# Autodesk Inventor assembly: Clutch Concept
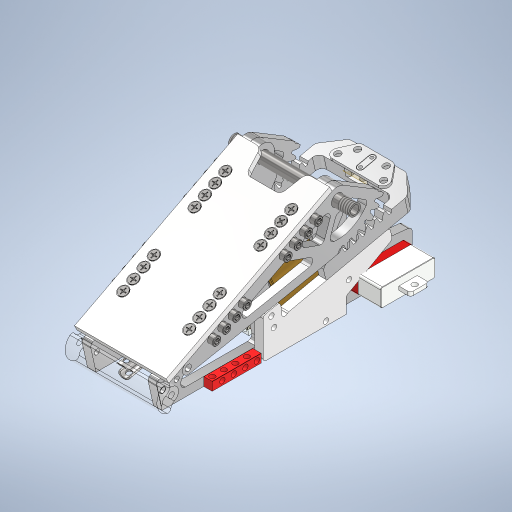
[picture p0: Inventor's stored thumbnail of the model, 512x512]
Saved by Autodesk Inventor 2023.4 (Build 274418000, 418)
## iProperties
Created: 2024-02-03
Part Number: Clutch Concept
Document SubType Name: Assembly
Designer: Nathan Cai
Mass: 1134.93 g
Surface Area: 3804.81 cm^2
Volume: 547.921 cm^3
Density: 2.07134 g/cm^3
Author: Nathan Cai
## Documents named in this file (35)
- E:\Documents\Inventor\Bleep V1.3\Clutch Concept.iam
- E:\Documents\Inventor\Bleep V1.3\Flywheel.ipt
- E:\Documents\Inventor\Bleep V1.3\Thrust Bearing.ipt
- E:\Documents\Inventor\Bleep V1.3\BB 13x19x4.ipt
- E:\Documents\Inventor\Bleep V1.3\Cup.ipt
- E:\Documents\Inventor\Bleep V1.3\1561T741_Stacked Wave Disc Spring\1561T741_Stacked Wave Disc Spring.ipt
- E:\Documents\Inventor\Bleep V1.3\AKK RS2205 2300KV\AKK RS2205 2300KV.iam
- E:\Documents\Inventor\Bleep V1.3\Nut Strip 2x1 - 4-40.ipt
- E:\Documents\Inventor\Bleep V1.3\BB 37mm x 30mm x 4mm.ipt
- E:\Documents\Inventor\Bleep V1.3\Motor Plate.ipt
- E:\Documents\Inventor\Bleep V1.3\Uprights.ipt
- E:\Documents\Inventor\Bleep V1.3\Nut Strip 4x4 - 4-40.ipt
- E:\Documents\Inventor\Bleep V1.3\5172T23_Metal Gear - 20 Degree Pressure Angle\5172T23_Metal Gear - 20 Degree Pressure Angle.ipt
- E:\Documents\Inventor\Bleep V1.3\BB .25x.5x.1875 - Flangeless.ipt
- E:\Documents\Inventor\Content Center Files\R2023\en-US\ANSI B18.3(13)\ANSI B18.3 - 4-40 UNC - 0.375(22).ipt
- E:\Documents\Inventor\Bleep V1.3\Lever.ipt
- E:\Documents\Inventor\Bleep V1.3\Part1\Part1.ipt
- E:\Documents\Inventor\Bleep V1.3\Cam - Lever.ipt
- E:\Documents\Inventor\Bleep V1.3\Cam - Shell.ipt
- E:\Documents\Inventor\Bleep V1.3\BB 3x7x3.ipt
- E:\Documents\Inventor\Bleep V1.3\Ramp.ipt
- E:\Documents\Inventor\Bleep V1.3\Lever - Copy.ipt
- E:\Documents\Inventor\Bleep V1.3\Brace.ipt
- E:\Documents\Inventor\Bleep V1.3\BB 3x7x3 - Copy.ipt
- E:\Documents\Inventor\Bleep V1.3\Shaft - Arms.ipt
- E:\Documents\Inventor\Bleep V1.3\Shaft - Flywheel C.ipt
- E:\Documents\Inventor\Bleep V1.3\Clutch C.ipt
- E:\Documents\Inventor\Bleep V1.3\Spring Mount.ipt
- E:\Documents\Inventor\Bleep V1.3\Spring Spool.ipt
- E:\Documents\Inventor\Bleep V1.3\Collar.ipt
- E:\Documents\Inventor\Content Center Files\R2023\en-US\ANSI B18.6.3(12)\ANSI B18.6.3 - 4-40 UNC - 0.375(15_).ipt
- E:\Documents\Inventor\Bleep V1.3\Front Bumper.ipt
- E:\Documents\Inventor\Bleep V1.3\Rack - Slot.ipt
- E:\Documents\Inventor\Bleep V1.3\Pin Cap - Slot.ipt
- E:\Documents\Inventor\Bleep V1.3\Export\STL\Lever Spacer.ipt
## Components (85 placed, 34 different names)
1. Front Bumper:1 — Angle:5, Mate:464, Mate:465
2. Pin Cap - Slot:1 — Mate:459, Mate:460, Mate:461
3. Lever Spacer:1 — Mate:462, Mate:463
4. Flywheel:1 — Mate:37, Flush:102, Mate:104, Mate:105, Mate:275, Mate:309
5. Shaft - Flywheel C:1 — Mate:306, Mate:307, Mate:308, Mate:310, Mate:311, Mate:312, Mate:313, Mate:314, Mate:315, Angle:4, Mate:319, Mate:321, Mate:324
6. Shaft - Arms:1 — Mate:257, Flush:118
7. Clutch C:1 — Mate:308, Angle:4
8. Rack - Slot:1 — Angle:1, Angle:3, Rotation/Translation:1, Mate:315, Mate:313, Mate:314, Mate:459, Mate:460, Mate:461
9. Cup:1 — Mate:26, Mate:27, Angle:1, Tangent:1
10. AKK RS2205 2300KV:1 [sub-assembly] — Mate:37, Flush:102, Mate:426
11. Motor Plate:1 — Mate:106, Mate:107, Mate:128, Mate:129, Mate:131, Mate:132, Mate:134, Mate:136, Flush:106, Mate:144, Mate:145, Mate:146, Mate:147, Mate:148, Mate:149, Mate:150, Mate:151, Mate:152, Mate:153, Mate:154, Mate:155, Mate:156, Mate:157, Mate:158, Mate:159, Flush:149, Mate:426
12. 1561T741_Stacked Wave Disc Spring:1 — Mate:311, Mate:312
13. Spring Mount:1 — Mate:316, Flush:149, Mate:317, Mate:320
14. Thrust Bearing:1 — Mate:319, Mate:320, Mate:322
15. Spring Spool:1 — Mate:321, Mate:322, Mate:325
16. Collar:1 — Mate:324, Mate:325
17. Uprights:1 — Mate:128, Mate:130, Flush:103, Flush:104, Mate:133, Mate:138, Mate:141, Flush:107, Mate:168, Mate:169, Mate:229, Mate:230, Flush:110, Mate:257, Mate:266, Mate:267, Mate:268, Mate:269, Flush:125, Mate:317, Mate:289, Mate:363, Angle:6, Angle:7
18. Uprights:2 — Flush:103, Mate:132, Flush:104, Mate:135, Mate:137, Mate:139, Mate:140, Mate:226, Mate:228, Flush:111, Mate:263, Mate:264, Mate:270, Mate:271, Flush:124, Mate:292, Mate:362, Angle:5, Mate:464, Mate:465, Mate:466, Mate:467, Mate:468
19. Brace:1 — Mate:226, Mate:228, Flush:111, Mate:292
20. Brace:2 — Mate:229, Mate:230, Flush:110, Mate:289
21. Nut Strip 4x4 - 4-40:1 — Mate:129, Mate:130, Mate:131, Mate:133, Mate:316
22. Nut Strip 4x4 - 4-40:2 — Mate:134, Mate:135, Mate:136, Mate:137
23. 5172T23_Metal Gear - 20 Degree Pressure Angle:1 — Mate:138, Mate:141, Flush:105, Angle:3, Mate:198, Mate:199, Mate:200, Mate:201, Mate:202, Mate:203, Mate:204, Rotation/Translation:1, Flush:118, Mate:369, Mate:427, Mate:428, Mate:429, Mate:430, Mate:431, Mate:432, Mate:433, Mate:434, Mate:435, Mate:436, Mate:437, Mate:438, Mate:439, Mate:440, Mate:441, Mate:442
24. 5172T23_Metal Gear - 20 Degree Pressure Angle:2 — Mate:139, Mate:140, Flush:105, Mate:192, Mate:193, Mate:194, Mate:195, Mate:196, Mate:197, Flush:150, Mate:443, Mate:444, Mate:445, Mate:446, Mate:447, Mate:448, Mate:449, Mate:450, Mate:451, Mate:452, Mate:453, Mate:454, Mate:455, Mate:456, Mate:457, Mate:458
25. BB .25x.5x.1875 - Flangeless:1 — Flush:106, Mate:310
26. Lever:1 — Mate:168, Mate:169, Tangent:1, Mate:181, Mate:182, Mate:190, Mate:326
27. Lever - Copy:1
28. Part1:1 — Mate:179, Mate:180, Angle:6, Angle:7, Mate:466, Mate:467, Mate:468
29. Cam - Lever:1 — Mate:177, Mate:178
30. Cam - Shell:1 — Mate:177, Mate:178, Mate:179, Mate:180
31. BB 3x7x3:1 — Mate:181, Mate:182
32. BB 3x7x3:2 — Mate:462, Mate:463
33. BB 3x7x3 - Copy:1 — Mate:190, Mate:326
34. BB 13x19x4:1 — Mate:26, Mate:27
35. BB 37mm x 30mm x 4mm:1 — Mate:104, Mate:105, Mate:106, Mate:107
36. BB .25x.5x.1875 - Flangeless:2 — Mate:275, Mate:306, Mate:307, Mate:309
37. Ramp:1 — Mate:204, Flush:150, Mate:369, Mate:370, Mate:371, Mate:372, Mate:373, Mate:374, Mate:375, Mate:376, Mate:377, Mate:378, Mate:379, Mate:380, Mate:381, Mate:382, Mate:383, Mate:384, Mate:385
38. Nut Strip 4x4 - 4-40:3 — Mate:192, Mate:193, Mate:194
39. Nut Strip 4x4 - 4-40:5 — Mate:199, Mate:200, Mate:201
40. Nut Strip 4x4 - 4-40:6 — Mate:198, Mate:202, Mate:203
41. Nut Strip 4x4 - 4-40:7 — Mate:195, Mate:196, Mate:197
42. Nut Strip 4x4 - 4-40:8 — Mate:266, Mate:267, Mate:363
43. Nut Strip 4x4 - 4-40:9 — Mate:263, Mate:264, Mate:362
44. Nut Strip 2x1 - 4-40:3 — Mate:270, Mate:271, Flush:124
45. Nut Strip 2x1 - 4-40:4 — Mate:268, Mate:269, Flush:125
46. Spline Socket Head Cap Screw - Inch 4-40 UNC - 0.375:9 — Mate:427, Mate:428
47. Spline Socket Head Cap Screw - Inch 4-40 UNC - 0.375:10 — Mate:429, Mate:430
48. Spline Socket Head Cap Screw - Inch 4-40 UNC - 0.375:11 — Mate:431, Mate:432
49. Spline Socket Head Cap Screw - Inch 4-40 UNC - 0.375:12 — Mate:433, Mate:434
50. Spline Socket Head Cap Screw - Inch 4-40 UNC - 0.375:13 — Mate:435, Mate:436
51. Spline Socket Head Cap Screw - Inch 4-40 UNC - 0.375:14 — Mate:437, Mate:438
52. Spline Socket Head Cap Screw - Inch 4-40 UNC - 0.375:15 — Mate:439, Mate:440
53. Spline Socket Head Cap Screw - Inch 4-40 UNC - 0.375:16 — Mate:441, Mate:442
54. Spline Socket Head Cap Screw - Inch 4-40 UNC - 0.375:17 — Mate:443, Mate:444
55. Spline Socket Head Cap Screw - Inch 4-40 UNC - 0.375:18 — Mate:445, Mate:446
56. Spline Socket Head Cap Screw - Inch 4-40 UNC - 0.375:19 — Mate:447, Mate:448
57. Spline Socket Head Cap Screw - Inch 4-40 UNC - 0.375:20 — Mate:449, Mate:450
58. Spline Socket Head Cap Screw - Inch 4-40 UNC - 0.375:21 — Mate:451, Mate:452
59. Spline Socket Head Cap Screw - Inch 4-40 UNC - 0.375:22 — Mate:453, Mate:454
60. Spline Socket Head Cap Screw - Inch 4-40 UNC - 0.375:23 — Mate:455, Mate:456
61. Spline Socket Head Cap Screw - Inch 4-40 UNC - 0.375:24 — Mate:457, Mate:458
62. Cross Recessed Flat Countersunk Head Machine Screw - Type I - Inch 4-40 x 3/8:1 — Mate:370
63. Cross Recessed Flat Countersunk Head Machine Screw - Type I - Inch 4-40 x 3/8:2 — Mate:371
64. Cross Recessed Flat Countersunk Head Machine Screw - Type I - Inch 4-40 x 3/8:3 — Mate:372
65. Cross Recessed Flat Countersunk Head Machine Screw - Type I - Inch 4-40 x 3/8:4 — Mate:373
66. Cross Recessed Flat Countersunk Head Machine Screw - Type I - Inch 4-40 x 3/8:5 — Mate:374
67. Cross Recessed Flat Countersunk Head Machine Screw - Type I - Inch 4-40 x 3/8:6 — Mate:375
68. Cross Recessed Flat Countersunk Head Machine Screw - Type I - Inch 4-40 x 3/8:7 — Mate:376
69. Cross Recessed Flat Countersunk Head Machine Screw - Type I - Inch 4-40 x 3/8:8 — Mate:377
70. Cross Recessed Flat Countersunk Head Machine Screw - Type I - Inch 4-40 x 3/8:9 — Mate:378
71. Cross Recessed Flat Countersunk Head Machine Screw - Type I - Inch 4-40 x 3/8:10 — Mate:379
72. Cross Recessed Flat Countersunk Head Machine Screw - Type I - Inch 4-40 x 3/8:11 — Mate:380
73. Cross Recessed Flat Countersunk Head Machine Screw - Type I - Inch 4-40 x 3/8:12 — Mate:381
74. Cross Recessed Flat Countersunk Head Machine Screw - Type I - Inch 4-40 x 3/8:13 — Mate:382
75. Cross Recessed Flat Countersunk Head Machine Screw - Type I - Inch 4-40 x 3/8:14 — Mate:383
76. Cross Recessed Flat Countersunk Head Machine Screw - Type I - Inch 4-40 x 3/8:15 — Mate:384
77. Cross Recessed Flat Countersunk Head Machine Screw - Type I - Inch 4-40 x 3/8:16 — Mate:385
78. Spline Socket Head Cap Screw - Inch 4-40 UNC - 0.375:1 — Mate:144, Mate:145
79. Spline Socket Head Cap Screw - Inch 4-40 UNC - 0.375:2 — Mate:146, Mate:147
80. Spline Socket Head Cap Screw - Inch 4-40 UNC - 0.375:3 — Mate:148, Mate:149
81. Spline Socket Head Cap Screw - Inch 4-40 UNC - 0.375:4 — Mate:150, Mate:151
82. Spline Socket Head Cap Screw - Inch 4-40 UNC - 0.375:5 — Mate:152, Mate:153
83. Spline Socket Head Cap Screw - Inch 4-40 UNC - 0.375:6 — Mate:154, Mate:155
84. Spline Socket Head Cap Screw - Inch 4-40 UNC - 0.375:7 — Mate:156, Mate:157
85. Spline Socket Head Cap Screw - Inch 4-40 UNC - 0.375:8 — Mate:158, Mate:159
## Relationships (184: Mate 163, Flush 13, Angle 6, Tangent 1, RelateRotateTranslate 1)
- [Mate]: Clutch C:1 ↔ BB 13x19x4:1
- [Mate]: Clutch C:1 ↔ BB 13x19x4:1
- Mate:26: Cup:1 ↔ BB 13x19x4:1
- Mate:27: Cup:1 ↔ BB 13x19x4:1
- Mate:37: Flywheel:1 ↔ AKK RS2205 2300KV:1
- Angle:1 (0 deg): Rack - Slot:1 ↔ Cup:1
- Flush:102: Flywheel:1 ↔ AKK RS2205 2300KV:1
- Mate:104: Flywheel:1 ↔ BB 37mm x 30mm x 4mm:1
- Mate:105: Flywheel:1 ↔ BB 37mm x 30mm x 4mm:1
- Mate:106: Motor Plate:1 ↔ BB 37mm x 30mm x 4mm:1
- Mate:107: Motor Plate:1 ↔ BB 37mm x 30mm x 4mm:1
- Mate:128: Motor Plate:1 ↔ Uprights:1
- Mate:129: Motor Plate:1 ↔ Nut Strip 4x4 - 4-40:1
- Mate:130: Uprights:1 ↔ Nut Strip 4x4 - 4-40:1
- Mate:131: Motor Plate:1 ↔ Nut Strip 4x4 - 4-40:1
- Flush:103: Uprights:1 ↔ Uprights:2
- Mate:132: Motor Plate:1 ↔ Uprights:2
- Flush:104: Uprights:1 ↔ Uprights:2
- Mate:133: Uprights:1 ↔ Nut Strip 4x4 - 4-40:1
- Mate:134: Motor Plate:1 ↔ Nut Strip 4x4 - 4-40:2
- Mate:135: Uprights:2 ↔ Nut Strip 4x4 - 4-40:2
- Mate:136: Motor Plate:1 ↔ Nut Strip 4x4 - 4-40:2
- Mate:137: Uprights:2 ↔ Nut Strip 4x4 - 4-40:2
- Mate:138: Uprights:1 ↔ 5172T23_Metal Gear - 20 Degree Pressure Angle:1
- Mate:139: Uprights:2 ↔ 5172T23_Metal Gear - 20 Degree Pressure Angle:2
- Mate:140: Uprights:2 ↔ 5172T23_Metal Gear - 20 Degree Pressure Angle:2
- Mate:141: Uprights:1 ↔ 5172T23_Metal Gear - 20 Degree Pressure Angle:1
- Flush:105: 5172T23_Metal Gear - 20 Degree Pressure Angle:1 ↔ 5172T23_Metal Gear - 20 Degree Pressure Angle:2
- Flush:106: Motor Plate:1 ↔ BB .25x.5x.1875 - Flangeless:1
- Mate:144: Motor Plate:1 ↔ Spline Socket Head Cap Screw - Inch 4-40 UNC - 0.375:1
- Mate:145: Motor Plate:1 ↔ Spline Socket Head Cap Screw - Inch 4-40 UNC - 0.375:1
- Mate:146: Motor Plate:1 ↔ Spline Socket Head Cap Screw - Inch 4-40 UNC - 0.375:2
- Mate:147: Motor Plate:1 ↔ Spline Socket Head Cap Screw - Inch 4-40 UNC - 0.375:2
- Mate:148: Motor Plate:1 ↔ Spline Socket Head Cap Screw - Inch 4-40 UNC - 0.375:3
- Mate:149: Motor Plate:1 ↔ Spline Socket Head Cap Screw - Inch 4-40 UNC - 0.375:3
- Mate:150: Motor Plate:1 ↔ Spline Socket Head Cap Screw - Inch 4-40 UNC - 0.375:4
- Mate:151: Motor Plate:1 ↔ Spline Socket Head Cap Screw - Inch 4-40 UNC - 0.375:4
- Mate:152: Motor Plate:1 ↔ Spline Socket Head Cap Screw - Inch 4-40 UNC - 0.375:5
- Mate:153: Motor Plate:1 ↔ Spline Socket Head Cap Screw - Inch 4-40 UNC - 0.375:5
- Mate:154: Motor Plate:1 ↔ Spline Socket Head Cap Screw - Inch 4-40 UNC - 0.375:6
- Mate:155: Motor Plate:1 ↔ Spline Socket Head Cap Screw - Inch 4-40 UNC - 0.375:6
- Mate:156: Motor Plate:1 ↔ Spline Socket Head Cap Screw - Inch 4-40 UNC - 0.375:7
- Mate:157: Motor Plate:1 ↔ Spline Socket Head Cap Screw - Inch 4-40 UNC - 0.375:7
- Mate:158: Motor Plate:1 ↔ Spline Socket Head Cap Screw - Inch 4-40 UNC - 0.375:8
- Mate:159: Motor Plate:1 ↔ Spline Socket Head Cap Screw - Inch 4-40 UNC - 0.375:8
- Flush:107: Uprights:1
- Mate:168: Uprights:1 ↔ Lever:1
- Mate:169: Uprights:1 ↔ Lever:1
- Tangent:1: Cup:1 ↔ Lever:1
- Angle:3 (0 deg): Rack - Slot:1 ↔ 5172T23_Metal Gear - 20 Degree Pressure Angle:1
- [Mate]: Uprights:2 ↔ Lever - Copy:1
- [Mate]: Uprights:2 ↔ Lever - Copy:1
- [Mate]: Lever:1 ↔ Lever - Copy:1
- Mate:177: Cam - Lever:1 ↔ Cam - Shell:1
- Mate:178: Cam - Lever:1 ↔ Cam - Shell:1
- Mate:179: Part1:1 ↔ Cam - Shell:1
- Mate:180: Part1:1 ↔ Cam - Shell:1
- Mate:181: Lever:1 ↔ BB 3x7x3:1
- Mate:182: Lever:1 ↔ BB 3x7x3:1
- [Mate]: Lever - Copy:1 ↔ BB 3x7x3:2
- [Mate]: Lever - Copy:1 ↔ BB 3x7x3:2
- Mate:190: Lever:1 ↔ BB 3x7x3 - Copy:1
- Mate:192: 5172T23_Metal Gear - 20 Degree Pressure Angle:2 ↔ Nut Strip 4x4 - 4-40:3
- Mate:193: 5172T23_Metal Gear - 20 Degree Pressure Angle:2 ↔ Nut Strip 4x4 - 4-40:3
- Mate:194: 5172T23_Metal Gear - 20 Degree Pressure Angle:2 ↔ Nut Strip 4x4 - 4-40:3
- Mate:195: 5172T23_Metal Gear - 20 Degree Pressure Angle:2 ↔ Nut Strip 4x4 - 4-40:7
- Mate:196: 5172T23_Metal Gear - 20 Degree Pressure Angle:2 ↔ Nut Strip 4x4 - 4-40:7
- Mate:197: 5172T23_Metal Gear - 20 Degree Pressure Angle:2 ↔ Nut Strip 4x4 - 4-40:7
- Mate:198: 5172T23_Metal Gear - 20 Degree Pressure Angle:1 ↔ Nut Strip 4x4 - 4-40:6
- Mate:199: 5172T23_Metal Gear - 20 Degree Pressure Angle:1 ↔ Nut Strip 4x4 - 4-40:5
- Mate:200: 5172T23_Metal Gear - 20 Degree Pressure Angle:1 ↔ Nut Strip 4x4 - 4-40:5
- Mate:201: 5172T23_Metal Gear - 20 Degree Pressure Angle:1 ↔ Nut Strip 4x4 - 4-40:5
- Mate:202: 5172T23_Metal Gear - 20 Degree Pressure Angle:1 ↔ Nut Strip 4x4 - 4-40:6
- Mate:203: 5172T23_Metal Gear - 20 Degree Pressure Angle:1 ↔ Nut Strip 4x4 - 4-40:6
- Mate:204: 5172T23_Metal Gear - 20 Degree Pressure Angle:1 ↔ Ramp:1
- Flush:150: 5172T23_Metal Gear - 20 Degree Pressure Angle:2 ↔ Ramp:1
- Mate:226: Uprights:2 ↔ Brace:1
- Mate:228: Uprights:2 ↔ Brace:1
- Mate:229: Uprights:1 ↔ Brace:2
- Mate:230: Uprights:1 ↔ Brace:2
- Rotation/Translation:1 [RelateRotateTranslate] (159.5929 mm): Rack - Slot:1 ↔ 5172T23_Metal Gear - 20 Degree Pressure Angle:1
- Flush:110: Uprights:1 ↔ Brace:2
- Flush:111: Uprights:2 ↔ Brace:1
- Mate:257: Shaft - Arms:1 ↔ Uprights:1
- Flush:118 (-6.35 mm): Shaft - Arms:1 ↔ 5172T23_Metal Gear - 20 Degree Pressure Angle:1
- Mate:315 (31.75 mm): Shaft - Flywheel C:1 ↔ Rack - Slot:1
- Mate:263: Uprights:2 ↔ Nut Strip 4x4 - 4-40:9
- Mate:264: Uprights:2 ↔ Nut Strip 4x4 - 4-40:9
- Mate:266: Uprights:1 ↔ Nut Strip 4x4 - 4-40:8
- Mate:267: Uprights:1 ↔ Nut Strip 4x4 - 4-40:8
- Mate:268: Uprights:1 ↔ Nut Strip 2x1 - 4-40:4
- Mate:269: Uprights:1 ↔ Nut Strip 2x1 - 4-40:4
- Mate:270: Uprights:2 ↔ Nut Strip 2x1 - 4-40:3
- Mate:271: Uprights:2 ↔ Nut Strip 2x1 - 4-40:3
- Flush:124: Uprights:2 ↔ Nut Strip 2x1 - 4-40:3
- Flush:125: Uprights:1 ↔ Nut Strip 2x1 - 4-40:4
- Mate:275: Flywheel:1 ↔ BB .25x.5x.1875 - Flangeless:2
- Mate:289: Uprights:1 ↔ Brace:2
- Mate:292: Uprights:2 ↔ Brace:1
- Mate:306: Shaft - Flywheel C:1 ↔ BB .25x.5x.1875 - Flangeless:2
- Mate:307: Shaft - Flywheel C:1 ↔ BB .25x.5x.1875 - Flangeless:2
- Mate:308: Shaft - Flywheel C:1 ↔ Clutch C:1
- Mate:309: Flywheel:1 ↔ BB .25x.5x.1875 - Flangeless:2
- Mate:310: Shaft - Flywheel C:1 ↔ BB .25x.5x.1875 - Flangeless:1
- Mate:311: Shaft - Flywheel C:1 ↔ 1561T741_Stacked Wave Disc Spring:1
- Mate:312: Shaft - Flywheel C:1 ↔ 1561T741_Stacked Wave Disc Spring:1
- Mate:313: Shaft - Flywheel C:1 ↔ Rack - Slot:1
- Mate:314: Shaft - Flywheel C:1 ↔ Rack - Slot:1
- Angle:4 (0 deg): Shaft - Flywheel C:1 ↔ Clutch C:1
- Mate:316: Spring Mount:1 ↔ Nut Strip 4x4 - 4-40:1
- Flush:149 (2.3813 mm): Motor Plate:1 ↔ Spring Mount:1
- Mate:317: Spring Mount:1 ↔ Uprights:1
- Mate:319: Shaft - Flywheel C:1 ↔ Thrust Bearing:1
- Mate:320: Spring Mount:1 ↔ Thrust Bearing:1
- Mate:321: Shaft - Flywheel C:1 ↔ Spring Spool:1
- Mate:322: Thrust Bearing:1 ↔ Spring Spool:1
- Mate:324: Shaft - Flywheel C:1 ↔ Collar:1
- Mate:325: Spring Spool:1 ↔ Collar:1
- Mate:326: Lever:1 ↔ BB 3x7x3 - Copy:1
- Mate:362: Uprights:2 ↔ Nut Strip 4x4 - 4-40:9
- Mate:363: Uprights:1 ↔ Nut Strip 4x4 - 4-40:8
- Mate:369: 5172T23_Metal Gear - 20 Degree Pressure Angle:1 ↔ Ramp:1
- Mate:370: Ramp:1 ↔ Cross Recessed Flat Countersunk Head Machine Screw - Type I - Inch 4-40 x 3/8:1
- Mate:371: Ramp:1 ↔ Cross Recessed Flat Countersunk Head Machine Screw - Type I - Inch 4-40 x 3/8:2
- Mate:372: Ramp:1 ↔ Cross Recessed Flat Countersunk Head Machine Screw - Type I - Inch 4-40 x 3/8:3
- Mate:373: Ramp:1 ↔ Cross Recessed Flat Countersunk Head Machine Screw - Type I - Inch 4-40 x 3/8:4
- Mate:374: Ramp:1 ↔ Cross Recessed Flat Countersunk Head Machine Screw - Type I - Inch 4-40 x 3/8:5
- Mate:375: Ramp:1 ↔ Cross Recessed Flat Countersunk Head Machine Screw - Type I - Inch 4-40 x 3/8:6
- Mate:376: Ramp:1 ↔ Cross Recessed Flat Countersunk Head Machine Screw - Type I - Inch 4-40 x 3/8:7
- Mate:377: Ramp:1 ↔ Cross Recessed Flat Countersunk Head Machine Screw - Type I - Inch 4-40 x 3/8:8
- Mate:378: Ramp:1 ↔ Cross Recessed Flat Countersunk Head Machine Screw - Type I - Inch 4-40 x 3/8:9
- Mate:379: Ramp:1 ↔ Cross Recessed Flat Countersunk Head Machine Screw - Type I - Inch 4-40 x 3/8:10
- Mate:380: Ramp:1 ↔ Cross Recessed Flat Countersunk Head Machine Screw - Type I - Inch 4-40 x 3/8:11
- Mate:381: Ramp:1 ↔ Cross Recessed Flat Countersunk Head Machine Screw - Type I - Inch 4-40 x 3/8:12
- Mate:382: Ramp:1 ↔ Cross Recessed Flat Countersunk Head Machine Screw - Type I - Inch 4-40 x 3/8:13
- Mate:383: Ramp:1 ↔ Cross Recessed Flat Countersunk Head Machine Screw - Type I - Inch 4-40 x 3/8:14
- Mate:384: Ramp:1 ↔ Cross Recessed Flat Countersunk Head Machine Screw - Type I - Inch 4-40 x 3/8:15
- Mate:385: Ramp:1 ↔ Cross Recessed Flat Countersunk Head Machine Screw - Type I - Inch 4-40 x 3/8:16
- Angle:5 (180 deg): Front Bumper:1 ↔ Uprights:2
- Mate:426: AKK RS2205 2300KV:1 ↔ Motor Plate:1
- Mate:427: 5172T23_Metal Gear - 20 Degree Pressure Angle:1 ↔ Spline Socket Head Cap Screw - Inch 4-40 UNC - 0.375:9
- Mate:428: 5172T23_Metal Gear - 20 Degree Pressure Angle:1 ↔ Spline Socket Head Cap Screw - Inch 4-40 UNC - 0.375:9
- Mate:429: 5172T23_Metal Gear - 20 Degree Pressure Angle:1 ↔ Spline Socket Head Cap Screw - Inch 4-40 UNC - 0.375:10
- Mate:430: 5172T23_Metal Gear - 20 Degree Pressure Angle:1 ↔ Spline Socket Head Cap Screw - Inch 4-40 UNC - 0.375:10
- Mate:431: 5172T23_Metal Gear - 20 Degree Pressure Angle:1 ↔ Spline Socket Head Cap Screw - Inch 4-40 UNC - 0.375:11
- Mate:432: 5172T23_Metal Gear - 20 Degree Pressure Angle:1 ↔ Spline Socket Head Cap Screw - Inch 4-40 UNC - 0.375:11
- Mate:433: 5172T23_Metal Gear - 20 Degree Pressure Angle:1 ↔ Spline Socket Head Cap Screw - Inch 4-40 UNC - 0.375:12
- Mate:434: 5172T23_Metal Gear - 20 Degree Pressure Angle:1 ↔ Spline Socket Head Cap Screw - Inch 4-40 UNC - 0.375:12
- Mate:435: 5172T23_Metal Gear - 20 Degree Pressure Angle:1 ↔ Spline Socket Head Cap Screw - Inch 4-40 UNC - 0.375:13
- Mate:436: 5172T23_Metal Gear - 20 Degree Pressure Angle:1 ↔ Spline Socket Head Cap Screw - Inch 4-40 UNC - 0.375:13
- Mate:437: 5172T23_Metal Gear - 20 Degree Pressure Angle:1 ↔ Spline Socket Head Cap Screw - Inch 4-40 UNC - 0.375:14
- Mate:438: 5172T23_Metal Gear - 20 Degree Pressure Angle:1 ↔ Spline Socket Head Cap Screw - Inch 4-40 UNC - 0.375:14
- Mate:439: 5172T23_Metal Gear - 20 Degree Pressure Angle:1 ↔ Spline Socket Head Cap Screw - Inch 4-40 UNC - 0.375:15
- Mate:440: 5172T23_Metal Gear - 20 Degree Pressure Angle:1 ↔ Spline Socket Head Cap Screw - Inch 4-40 UNC - 0.375:15
- Mate:441: 5172T23_Metal Gear - 20 Degree Pressure Angle:1 ↔ Spline Socket Head Cap Screw - Inch 4-40 UNC - 0.375:16
- Mate:442: 5172T23_Metal Gear - 20 Degree Pressure Angle:1 ↔ Spline Socket Head Cap Screw - Inch 4-40 UNC - 0.375:16
- Mate:443: 5172T23_Metal Gear - 20 Degree Pressure Angle:2 ↔ Spline Socket Head Cap Screw - Inch 4-40 UNC - 0.375:17
- Mate:444: 5172T23_Metal Gear - 20 Degree Pressure Angle:2 ↔ Spline Socket Head Cap Screw - Inch 4-40 UNC - 0.375:17
- Mate:445: 5172T23_Metal Gear - 20 Degree Pressure Angle:2 ↔ Spline Socket Head Cap Screw - Inch 4-40 UNC - 0.375:18
- Mate:446: 5172T23_Metal Gear - 20 Degree Pressure Angle:2 ↔ Spline Socket Head Cap Screw - Inch 4-40 UNC - 0.375:18
- Mate:447: 5172T23_Metal Gear - 20 Degree Pressure Angle:2 ↔ Spline Socket Head Cap Screw - Inch 4-40 UNC - 0.375:19
- Mate:448: 5172T23_Metal Gear - 20 Degree Pressure Angle:2 ↔ Spline Socket Head Cap Screw - Inch 4-40 UNC - 0.375:19
- Mate:449: 5172T23_Metal Gear - 20 Degree Pressure Angle:2 ↔ Spline Socket Head Cap Screw - Inch 4-40 UNC - 0.375:20
- Mate:450: 5172T23_Metal Gear - 20 Degree Pressure Angle:2 ↔ Spline Socket Head Cap Screw - Inch 4-40 UNC - 0.375:20
- Mate:451: 5172T23_Metal Gear - 20 Degree Pressure Angle:2 ↔ Spline Socket Head Cap Screw - Inch 4-40 UNC - 0.375:21
- Mate:452: 5172T23_Metal Gear - 20 Degree Pressure Angle:2 ↔ Spline Socket Head Cap Screw - Inch 4-40 UNC - 0.375:21
- Mate:453: 5172T23_Metal Gear - 20 Degree Pressure Angle:2 ↔ Spline Socket Head Cap Screw - Inch 4-40 UNC - 0.375:22
- Mate:454: 5172T23_Metal Gear - 20 Degree Pressure Angle:2 ↔ Spline Socket Head Cap Screw - Inch 4-40 UNC - 0.375:22
- Mate:455: 5172T23_Metal Gear - 20 Degree Pressure Angle:2 ↔ Spline Socket Head Cap Screw - Inch 4-40 UNC - 0.375:23
- Mate:456: 5172T23_Metal Gear - 20 Degree Pressure Angle:2 ↔ Spline Socket Head Cap Screw - Inch 4-40 UNC - 0.375:23
- Mate:457: 5172T23_Metal Gear - 20 Degree Pressure Angle:2 ↔ Spline Socket Head Cap Screw - Inch 4-40 UNC - 0.375:24
- Mate:458: 5172T23_Metal Gear - 20 Degree Pressure Angle:2 ↔ Spline Socket Head Cap Screw - Inch 4-40 UNC - 0.375:24
- Mate:459: Pin Cap - Slot:1 ↔ Rack - Slot:1
- Mate:460: Pin Cap - Slot:1 ↔ Rack - Slot:1
- Mate:461: Pin Cap - Slot:1 ↔ Rack - Slot:1
- Mate:462: Lever Spacer:1 ↔ BB 3x7x3:2
- Mate:463: Lever Spacer:1 ↔ BB 3x7x3:2
- Angle:6 (180 deg): Uprights:1 ↔ Part1:1
- Angle:7 (0 deg): Uprights:1 ↔ Part1:1
- Mate:464: Front Bumper:1 ↔ Uprights:2
- Mate:465: Front Bumper:1 ↔ Uprights:2
- Mate:466: Uprights:2 ↔ Part1:1
- Mate:467: Uprights:2 ↔ Part1:1
- Mate:468: Uprights:2 ↔ Part1:1
